# Autodesk Inventor assembly: Metal Scoop
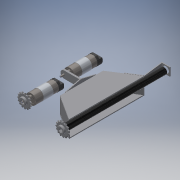
[picture p0: Inventor's stored thumbnail of the model, 180x180]
Saved by Autodesk Inventor 2017 (Build 210142000, 142)
## iProperties
Created: 2017-06-10
Part Number: Metal Scoop
Document SubType Name: Assembly
Designer: Matthew
Author: Matthew
## Documents named in this file (11)
- C:\Inventor Stuff\Robotics Trash\Metal Scoop\Metal Scoop.iam
- C:\Inventor Stuff\Robotics Trash\Metal Scoop\Top + Bottom.ipt
- C:\Inventor Stuff\Robotics Trash\Metal Scoop\Back Wall.ipt
- C:\Inventor Stuff\Robotics Trash\Metal Scoop\Side Wall.ipt
- C:\Inventor Stuff\Robotics Trash\Metal Scoop\Pivot Bracket.ipt
- C:\Inventor Stuff\Robotics Trash\Metal Scoop\Pivot Bracket Other Side.ipt
- C:\Inventor Stuff\Robotics Trash\Metal Scoop\Top + Spinner.ipt
- C:\Inventor Stuff\Robotics Trash\Tetrix Neverest 20 Motor.ipt
- C:\Inventor Stuff\Robotics Trash\VexPro 15 Tooth Sprocket.ipt
- C:\Inventor Stuff\Robotics Trash\Metal Scoop\Spinner to Top.ipt
- C:\Inventor Stuff\Robotics Trash\Metal Scoop\Pivot Bracket 2.ipt
## Components (14 placed, 10 different names)
1. Top + Bottom:1 — Mate:2, Flush:2, Mate:11, Mate:17, Flush:10, Mate:18, Mate:19, Flush:11
2. Back Wall:1 — Mate:2, Flush:2, Flush:4, Mate:10, Mate:11, Mate:12, Mate:13, Mate:14, Mate:15, Mate:16, Flush:12, Mate:21, Mate:28
3. Top + Bottom:2 — Flush:4, Flush:8, Flush:9, Mate:12, Mate:15, Mate:20
4. Pivot Bracket:1 — Flush:8, Mate:10, Mate:13
5. Pivot Bracket Other Side:1 — Flush:9, Mate:14, Mate:16
6. Side Wall:1 — Mate:17, Flush:10, Mate:18, Mate:22, Mate:31
7. Side Wall:2 — Mate:19, Flush:11, Mate:20, Mate:27
8. Top + Spinner:1 — Flush:12, Mate:21, Mate:22, Flush:13, Mate:25, Mate:26, Flush:15
9. Tetrix Neverest 20 Motor:2 — Flush:13, Mate:24
10. VexPro 15 Tooth Sprocket:1 — Mate:25, Flush:14
11. VexPro 15 Tooth Sprocket:2 — Mate:24, Flush:14
12. Spinner to Top:1 — Mate:26, Mate:27
13. Pivot Bracket 2:1 — Mate:28, Flush:15, Mate:29, Mate:30, Mate:31
14. Tetrix Neverest 20 Motor:3 — Mate:29, Mate:30
## Relationships (32: Mate 22, Flush 10)
- Mate:2: Top + Bottom:1 ↔ Back Wall:1
- Flush:2: Top + Bottom:1 ↔ Back Wall:1
- Flush:4: Back Wall:1 ↔ Top + Bottom:2
- Flush:8: Top + Bottom:2 ↔ Pivot Bracket:1
- Flush:9: Top + Bottom:2 ↔ Pivot Bracket Other Side:1
- Mate:10: Back Wall:1 ↔ Pivot Bracket:1
- Mate:11: Top + Bottom:1 ↔ Back Wall:1
- Mate:12: Back Wall:1 ↔ Top + Bottom:2
- Mate:13: Back Wall:1 ↔ Pivot Bracket:1
- Mate:14: Back Wall:1 ↔ Pivot Bracket Other Side:1
- Mate:15: Back Wall:1 ↔ Top + Bottom:2
- Mate:16: Back Wall:1 ↔ Pivot Bracket Other Side:1
- Mate:17: Top + Bottom:1 ↔ Side Wall:1
- Flush:10: Top + Bottom:1 ↔ Side Wall:1
- Mate:18: Top + Bottom:1 ↔ Side Wall:1
- Mate:19: Top + Bottom:1 ↔ Side Wall:2
- Flush:11: Top + Bottom:1 ↔ Side Wall:2
- Mate:20: Top + Bottom:2 ↔ Side Wall:2
- Flush:12: Back Wall:1 ↔ Top + Spinner:1
- Mate:21: Back Wall:1 ↔ Top + Spinner:1
- Mate:22: Side Wall:1 ↔ Top + Spinner:1
- Flush:13 (-12.7 mm): Top + Spinner:1 ↔ Tetrix Neverest 20 Motor:2
- Mate:24: Tetrix Neverest 20 Motor:2 ↔ VexPro 15 Tooth Sprocket:2
- Mate:25: Top + Spinner:1 ↔ VexPro 15 Tooth Sprocket:1
- Flush:14: VexPro 15 Tooth Sprocket:1 ↔ VexPro 15 Tooth Sprocket:2
- Mate:26: Top + Spinner:1 ↔ Spinner to Top:1
- Mate:27: Side Wall:2 ↔ Spinner to Top:1
- Mate:28: Back Wall:1 ↔ Pivot Bracket 2:1
- Flush:15 (-12.7 mm): Top + Spinner:1 ↔ Pivot Bracket 2:1
- Mate:29: Pivot Bracket 2:1 ↔ Tetrix Neverest 20 Motor:3
- Mate:30 (6.35 mm): Pivot Bracket 2:1 ↔ Tetrix Neverest 20 Motor:3
- Mate:31 (74.6125 mm): Side Wall:1 ↔ Pivot Bracket 2:1
